# Autodesk Inventor assembly: Drive-B Unit
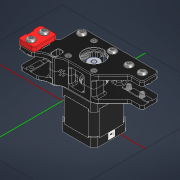
[picture p0: Inventor's stored thumbnail of the model, 180x180]
Saved by Autodesk Inventor 2022.2 (Build 262287010, 287A)
## iProperties
Created: 2022-03-14
Part Number: Drive-B Unit
Document SubType Name: Assembly
Designer: sleib
Author: sleib
## Documents named in this file (11)
- C:\Users\sleib\Projekte\Voron-2\CAD\Inventor\Drive-B Unit.iam
- C:\Users\sleib\Projekte\Voron-2\CAD\Inventor\Drive-B Frame.ipt
- C:\Users\sleib\Projekte\Voron-2\CAD\Inventor\NEMA17 Black.ipt
- C:\Users\sleib\Projekte\Voron-2\CAD\Inventor\M3x30 SHCS.ipt
- C:\Users\sleib\Projekte\Voron-2\CAD\Inventor\Z Belt-Clamp Upper.ipt
- C:\Users\sleib\Projekte\Voron-2\CAD\Inventor\M5x16 BHCS.ipt
- C:\Users\sleib\Projekte\Voron-2\CAD\Inventor\GT2 16T Pulley (6mm).ipt
- C:\Users\sleib\Projekte\Voron-2\CAD\Inventor\M5x10 BHCS.ipt
- C:\Users\sleib\Projekte\Voron-2\CAD\Inventor\M5 Spacer (1mm).ipt
- C:\Users\sleib\Projekte\Voron-2\CAD\Inventor\Bearing F695-ZZ.ipt
- C:\Users\sleib\Projekte\Voron-2\CAD\Inventor\M5x30 BHCS.ipt
## Components (27 placed, 10 different names)
1. Drive-B Frame:1 — Passend:1, Passend:2, Passend:3, Passend:4, Passend:5, Passend:6, Passend:8, Passend:12, Passend:13, Passend:14, Passend:15, Passend:18, Passend:19, Passend:22, Passend:24, Passend:25, Passend:26, Passend:27, Passend:28, Passend:29, Passend:30, Passend:31, Passend:32, Passend:40, Passend:41, Passend:42, Passend:58, Passend:59
2. NEMA17 Black:1 — Passend:9, Passend:10, Passend:11, Passend:15, Passend:23, Fluchtend:1
3. GT2 16T Pulley (6mm):1 — Passend:23, Fluchtend:1
4. Z Belt-Clamp Upper:1 — Passend:16, Passend:17, Passend:20, Passend:21, Passend:22
5. M3x30 SHCS:1 — Passend:6, Passend:10, Passend:13
6. M3x30 SHCS:2 — Passend:8, Passend:11, Passend:14
7. M3x30 SHCS:3 — Passend:5, Passend:9, Passend:12
8. M5x16 BHCS:1 — Passend:16, Passend:18, Passend:20
9. M5x16 BHCS:2 — Passend:17, Passend:19, Passend:21
10. M5x10 BHCS:1 — Passend:24, Passend:28
11. M5x10 BHCS:2 — Passend:25, Passend:29
12. M5x10 BHCS:3 — Passend:27, Passend:30
13. M5x10 BHCS:4 — Passend:26, Passend:31
14. M5 Spacer (1mm):1 — Passend:43, Passend:51
15. M5 Spacer (1mm):2 — Passend:46, Passend:53, Passend:54
16. M5 Spacer (1mm):3 — Passend:47, Passend:54, Passend:55
17. M5 Spacer (1mm):4 — Passend:48, Passend:57, Passend:58
18. M5 Spacer (1mm):5 — Passend:33, Passend:37
19. M5 Spacer (1mm):6 — Passend:36, Passend:39, Passend:41
20. Bearing F695-ZZ:1 — Passend:44, Passend:51, Passend:52
21. Bearing F695-ZZ:2 — Passend:45, Passend:52, Passend:53
22. Bearing F695-ZZ:3 — Passend:49, Passend:55, Passend:56
23. Bearing F695-ZZ:4 — Passend:50, Passend:56, Passend:57
24. Bearing F695-ZZ:5 — Passend:34, Passend:37, Passend:38
25. Bearing F695-ZZ:6 — Passend:35, Passend:38, Passend:39
26. M5x30 BHCS:1 — Passend:42, Passend:43, Passend:44, Passend:45, Passend:46, Passend:47, Passend:48, Passend:49, Passend:50, Passend:59
27. M5x30 BHCS:2 — Passend:32, Passend:33, Passend:34, Passend:35, Passend:36, Passend:40
## Relationships (59: Mate 58, Flush 1)
- Passend:1 [Mate]: Drive-B Frame:1
- Passend:2 [Mate]: Drive-B Frame:1
- Passend:3 [Mate]: Drive-B Frame:1
- Passend:4 [Mate]: Drive-B Frame:1
- Passend:5 [Mate]: Drive-B Frame:1 ↔ M3x30 SHCS:3
- Passend:6 [Mate]: Drive-B Frame:1 ↔ M3x30 SHCS:1
- Passend:8 [Mate]: Drive-B Frame:1 ↔ M3x30 SHCS:2
- Passend:9 [Mate]: NEMA17 Black:1 ↔ M3x30 SHCS:3
- Passend:10 [Mate]: NEMA17 Black:1 ↔ M3x30 SHCS:1
- Passend:11 [Mate]: NEMA17 Black:1 ↔ M3x30 SHCS:2
- Passend:12 [Mate]: Drive-B Frame:1 ↔ M3x30 SHCS:3
- Passend:13 [Mate]: Drive-B Frame:1 ↔ M3x30 SHCS:1
- Passend:14 [Mate]: Drive-B Frame:1 ↔ M3x30 SHCS:2
- Passend:15 [Mate]: Drive-B Frame:1 ↔ NEMA17 Black:1
- Passend:16 [Mate]: Z Belt-Clamp Upper:1 ↔ M5x16 BHCS:1
- Passend:17 [Mate]: Z Belt-Clamp Upper:1 ↔ M5x16 BHCS:2
- Passend:18 [Mate]: Drive-B Frame:1 ↔ M5x16 BHCS:1
- Passend:19 [Mate]: Drive-B Frame:1 ↔ M5x16 BHCS:2
- Passend:20 [Mate]: Z Belt-Clamp Upper:1 ↔ M5x16 BHCS:1
- Passend:21 [Mate]: Z Belt-Clamp Upper:1 ↔ M5x16 BHCS:2
- Passend:22 [Mate]: Drive-B Frame:1 ↔ Z Belt-Clamp Upper:1
- Passend:23 [Mate]: NEMA17 Black:1 ↔ GT2 16T Pulley (6mm):1
- Fluchtend:1 [Flush]: NEMA17 Black:1 ↔ GT2 16T Pulley (6mm):1
- Passend:24 [Mate]: Drive-B Frame:1 ↔ M5x10 BHCS:1
- Passend:25 [Mate]: Drive-B Frame:1 ↔ M5x10 BHCS:2
- Passend:26 [Mate]: Drive-B Frame:1 ↔ M5x10 BHCS:4
- Passend:27 [Mate]: Drive-B Frame:1 ↔ M5x10 BHCS:3
- Passend:28 [Mate]: Drive-B Frame:1 ↔ M5x10 BHCS:1
- Passend:29 [Mate]: Drive-B Frame:1 ↔ M5x10 BHCS:2
- Passend:30 [Mate]: Drive-B Frame:1 ↔ M5x10 BHCS:3
- Passend:31 [Mate]: Drive-B Frame:1 ↔ M5x10 BHCS:4
- Passend:32 [Mate]: Drive-B Frame:1 ↔ M5x30 BHCS:2
- Passend:33 [Mate]: M5 Spacer (1mm):5 ↔ M5x30 BHCS:2
- Passend:34 [Mate]: Bearing F695-ZZ:5 ↔ M5x30 BHCS:2
- Passend:35 [Mate]: Bearing F695-ZZ:6 ↔ M5x30 BHCS:2
- Passend:36 [Mate]: M5 Spacer (1mm):6 ↔ M5x30 BHCS:2
- Passend:37 [Mate]: M5 Spacer (1mm):5 ↔ Bearing F695-ZZ:5
- Passend:38 [Mate]: Bearing F695-ZZ:5 ↔ Bearing F695-ZZ:6
- Passend:39 [Mate]: M5 Spacer (1mm):6 ↔ Bearing F695-ZZ:6
- Passend:40 [Mate]: Drive-B Frame:1 ↔ M5x30 BHCS:2
- Passend:41 [Mate]: Drive-B Frame:1 ↔ M5 Spacer (1mm):6
- Passend:42 [Mate]: Drive-B Frame:1 ↔ M5x30 BHCS:1
- Passend:43 [Mate]: M5 Spacer (1mm):1 ↔ M5x30 BHCS:1
- Passend:44 [Mate]: Bearing F695-ZZ:1 ↔ M5x30 BHCS:1
- Passend:45 [Mate]: Bearing F695-ZZ:2 ↔ M5x30 BHCS:1
- Passend:46 [Mate]: M5 Spacer (1mm):2 ↔ M5x30 BHCS:1
- Passend:47 [Mate]: M5 Spacer (1mm):3 ↔ M5x30 BHCS:1
- Passend:48 [Mate]: M5 Spacer (1mm):4 ↔ M5x30 BHCS:1
- Passend:49 [Mate]: Bearing F695-ZZ:3 ↔ M5x30 BHCS:1
- Passend:50 [Mate]: Bearing F695-ZZ:4 ↔ M5x30 BHCS:1
- Passend:51 [Mate]: M5 Spacer (1mm):1 ↔ Bearing F695-ZZ:1
- Passend:52 [Mate]: Bearing F695-ZZ:1 ↔ Bearing F695-ZZ:2
- Passend:53 [Mate]: M5 Spacer (1mm):2 ↔ Bearing F695-ZZ:2
- Passend:54 [Mate]: M5 Spacer (1mm):2 ↔ M5 Spacer (1mm):3
- Passend:55 [Mate]: M5 Spacer (1mm):3 ↔ Bearing F695-ZZ:3
- Passend:56 [Mate]: Bearing F695-ZZ:3 ↔ Bearing F695-ZZ:4
- Passend:57 [Mate]: M5 Spacer (1mm):4 ↔ Bearing F695-ZZ:4
- Passend:58 [Mate]: Drive-B Frame:1 ↔ M5 Spacer (1mm):4
- Passend:59 [Mate]: Drive-B Frame:1 ↔ M5x30 BHCS:1
